# Autodesk Inventor assembly: Assembly
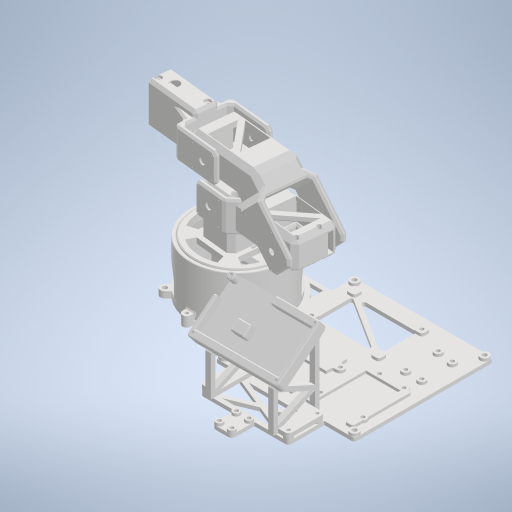
[picture p0: Inventor's stored thumbnail of the model, 512x512]
Saved by Autodesk Inventor 2023 (Build 270158000, 158)
## iProperties
Created: 2025-02-06
Part Number: Assembly
Document SubType Name: Assembly
Designer: Swoby
Author: Swoby
## Documents named in this file (13)
- C:\Users\Swoby\OneDrive\Plocha\DUM-E\V0.3\Light_model\Assembly.iam
- C:\Users\Swoby\OneDrive\Plocha\DUM-E\V0.3\Light_model\Base_BaseCircular.ipt
- C:\Users\Swoby\OneDrive\Plocha\DUM-E\V0.3\Light_model\Base_BasePlate.ipt
- C:\Users\Swoby\OneDrive\Plocha\DUM-E\V0.3\Light_model\Base_MotorHolder_L.ipt
- C:\Users\Swoby\OneDrive\Plocha\DUM-E\V0.3\Light_model\Base_MotorHolder_R.ipt
- C:\Users\Swoby\OneDrive\Plocha\DUM-E\V0.3\Light_model\Base_BaseCap.ipt
- C:\Users\Swoby\OneDrive\Plocha\DUM-E\V0.3\Light_model\Base_BaseCapCap.ipt
- C:\Users\Swoby\OneDrive\Plocha\DUM-E\V0.3\Light_model\Arm_1_Whole.ipt
- C:\Users\Swoby\OneDrive\Plocha\DUM-E\V0.3\Light_model\Arm_2_Whole.ipt
- C:\Users\Swoby\OneDrive\Plocha\DUM-E\V0.3\Light_model\Arm_3_Whole.ipt
- C:\Users\Swoby\OneDrive\Plocha\DUM-E\V0.3\Light_model\Base_ScreenHolder_L.ipt
- C:\Users\Swoby\OneDrive\Plocha\DUM-E\V0.3\Light_model\Base_ScreenHolder_R.ipt
- C:\Users\Swoby\OneDrive\Plocha\DUM-E\V0.3\Light_model\Base_ScreenHolder_Up.ipt
## Components (12 placed, 12 different names)
1. Base_BaseCircular:1 — Mate:1, Mate:2, Mate:5, Mate:7, Mate:8, Mate:13
2. Base_BasePlate:1 — Mate:1, Mate:2, Mate:4, Mate:9, Mate:10, Mate:11, Mate:12, Mate:13, Mate:14, Mate:27, Mate:28, Mate:29, Mate:33, Mate:34, Mate:35
3. Base_MotorHolder_L:1 — Mate:3, Flush:1, Flush:2, Mate:4
4. Base_MotorHolder_R:1 — Mate:3, Flush:1, Flush:2, Mate:5, Mate:14
5. Base_BaseCap:1 — Flush:3, Mate:6, Flush:4, Mate:7, Mate:8, Mate:15, Mate:16
6. Base_BaseCapCap:1 — Flush:3, Mate:6, Flush:4
7. Arm_1_Whole:1 — Mate:15, Mate:16, Mate:20, Mate:21
8. Arm_2_Whole:1 — Mate:20, Mate:21, Mate:22, Mate:23
9. Arm_3_Whole:1 — Mate:22, Mate:23
10. Base_ScreenHolder_L:1 — Mate:27, Mate:28, Mate:29, Mate:30, Mate:31, Mate:36
11. Base_ScreenHolder_R:1 — Mate:33, Mate:34, Mate:35
12. Base_ScreenHolder_Up:1 — Mate:30, Mate:31, Mate:36
## Relationships (33: Mate 29, Flush 4)
- Mate:1: Base_BaseCircular:1 ↔ Base_BasePlate:1
- Mate:2: Base_BaseCircular:1 ↔ Base_BasePlate:1
- Mate:3: Base_MotorHolder_L:1 ↔ Base_MotorHolder_R:1
- Flush:1: Base_MotorHolder_L:1 ↔ Base_MotorHolder_R:1
- Flush:2: Base_MotorHolder_L:1 ↔ Base_MotorHolder_R:1
- Mate:4: Base_BasePlate:1 ↔ Base_MotorHolder_L:1
- Mate:5: Base_BaseCircular:1 ↔ Base_MotorHolder_R:1
- Flush:3: Base_BaseCap:1 ↔ Base_BaseCapCap:1
- Mate:6: Base_BaseCap:1 ↔ Base_BaseCapCap:1
- Flush:4: Base_BaseCap:1 ↔ Base_BaseCapCap:1
- Mate:7: Base_BaseCircular:1 ↔ Base_BaseCap:1
- Mate:8: Base_BaseCircular:1 ↔ Base_BaseCap:1
- Mate:9: Base_BasePlate:1
- Mate:10: Base_BasePlate:1
- Mate:11: Base_BasePlate:1
- Mate:12: Base_BasePlate:1
- Mate:13: Base_BaseCircular:1 ↔ Base_BasePlate:1
- Mate:14: Base_BasePlate:1 ↔ Base_MotorHolder_R:1
- Mate:15: Base_BaseCap:1 ↔ Arm_1_Whole:1
- Mate:16 (1 mm): Base_BaseCap:1 ↔ Arm_1_Whole:1
- Mate:20: Arm_1_Whole:1 ↔ Arm_2_Whole:1
- Mate:21 (1 mm): Arm_1_Whole:1 ↔ Arm_2_Whole:1
- Mate:22: Arm_2_Whole:1 ↔ Arm_3_Whole:1
- Mate:23 (1 mm): Arm_2_Whole:1 ↔ Arm_3_Whole:1
- Mate:27: Base_BasePlate:1 ↔ Base_ScreenHolder_L:1
- Mate:28: Base_BasePlate:1 ↔ Base_ScreenHolder_L:1
- Mate:29: Base_BasePlate:1 ↔ Base_ScreenHolder_L:1
- Mate:30 (0.1 mm): Base_ScreenHolder_L:1 ↔ Base_ScreenHolder_Up:1
- Mate:31 (0.1 mm): Base_ScreenHolder_L:1 ↔ Base_ScreenHolder_Up:1
- Mate:33: Base_BasePlate:1 ↔ Base_ScreenHolder_R:1
- Mate:34: Base_BasePlate:1 ↔ Base_ScreenHolder_R:1
- Mate:35: Base_BasePlate:1 ↔ Base_ScreenHolder_R:1
- Mate:36: Base_ScreenHolder_L:1 ↔ Base_ScreenHolder_Up:1
